# Autodesk Inventor assembly: Clavicula
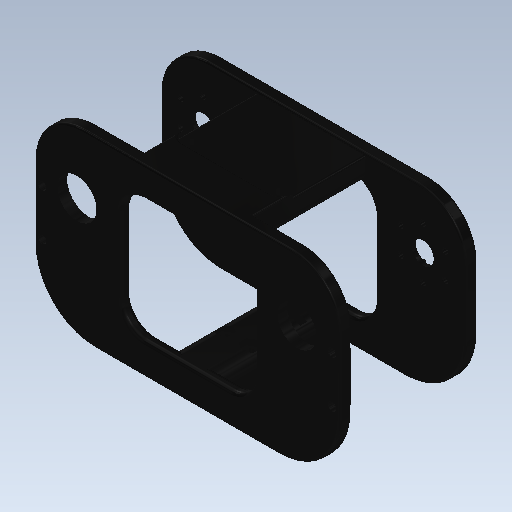
[picture p0: Inventor's stored thumbnail of the model, 512x512]
Saved by Autodesk Inventor 2020 (Build 240168000, 168)
## iProperties
Created: 2021-10-27
Part Number: Clavicula
Document SubType Name: Assembly
Designer: JCarlos
Author: JCarlos
## Documents named in this file (3)
- C:\Users\candu\Google Drive\Doutorado_UTFPR\Projeto_1_SpotMicro\Projeto_3D\Robo_Montado_v3\Clavicula.iam
- C:\Users\candu\Google Drive\Doutorado_UTFPR\Projeto_1_SpotMicro\Projeto_3D\Robo_Montado_v3\Estrutura_Corpo_Interno.ipt
- C:\Users\candu\Google Drive\Doutorado_UTFPR\Projeto_1_SpotMicro\Projeto_3D\Robo_Montado_v3\Fechamento_Corpo.ipt
## Components (2 placed, 2 different names)
1. Estrutura_Corpo_Interno:1 — Coincidência:1, Coincidência:2, Coincidência:3
2. Fechamento_Corpo:1 — Coincidência:1, Coincidência:2, Coincidência:3
## Relationships (3: Mate 3)
- Coincidência:1 [Mate]: Estrutura_Corpo_Interno:1 ↔ Fechamento_Corpo:1
- Coincidência:2 [Mate]: Estrutura_Corpo_Interno:1 ↔ Fechamento_Corpo:1
- Coincidência:3 [Mate]: Estrutura_Corpo_Interno:1 ↔ Fechamento_Corpo:1
